# Autodesk Inventor assembly: am-2256 4 in HiGrip Wheel_HexBore
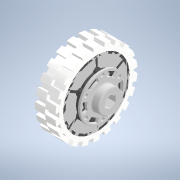
[picture p0: Inventor's stored thumbnail of the model, 180x180]
Saved by Autodesk Inventor 2020 (Build 240168000, 168)
## iProperties
Created: 2012-12-03
Part Number: am-2256 4 in HiGrip Wheel_HexBore
Description: STEP AP214
Document SubType Name: Assembly
Designer: srini
Sending System: SolidWorks 2010
Preprocessor: SwSTEP 2.0
Title: 4 in HiGrip Wheel.STEP
Revision Number: ANY
## Documents named in this file (5)
- C:\Users\srini\Documents\FRC\2020\am-2256 4 in HiGrip Wheel_HexBore.iam
- C:\Users\srini\Documents\FRC\2020\4in 2013 Hub.ipt
- C:\Users\srini\Documents\FRC\2020\4 in tread.ipt
- C:\Users\srini\Documents\FRC\2020\WheelMod4.ipt
- C:\Users\srini\Documents\FRC\2020\1_2_Hex_Bore_Aluminum_VersaHub_217-2592.ipt
## Components (6 placed, 4 different names)
1. 4in 2013 Hub_1 — Insert:1, Insert:2, Insert:3, Insert:4
2. 4 in tread_2 — Flush:1
3. WheelMod4:1 — Flush:1
4. 1_2_Hex_Bore_Aluminum_VersaHub_217-2592:1 — Insert:1, Insert:2
5. 1_2_Hex_Bore_Aluminum_VersaHub_217-2592:2 — Insert:3, Insert:4, Insert:5
6. 1_2_Hex_Bore_Aluminum_VersaHub_217-2592:3 — Insert:5
## Relationships (6: Insert 5, Flush 1)
- Flush:1: 4 in tread_2 ↔ WheelMod4:1
- Insert:1: 4in 2013 Hub_1 ↔ 1_2_Hex_Bore_Aluminum_VersaHub_217-2592:1
- Insert:2: 4in 2013 Hub_1 ↔ 1_2_Hex_Bore_Aluminum_VersaHub_217-2592:1
- Insert:3: 4in 2013 Hub_1 ↔ 1_2_Hex_Bore_Aluminum_VersaHub_217-2592:2
- Insert:4: 4in 2013 Hub_1 ↔ 1_2_Hex_Bore_Aluminum_VersaHub_217-2592:2
- Insert:5: 1_2_Hex_Bore_Aluminum_VersaHub_217-2592:2 ↔ 1_2_Hex_Bore_Aluminum_VersaHub_217-2592:3
